# Autodesk Inventor assembly: 23-004
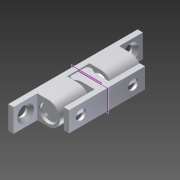
[picture p0: Inventor's stored thumbnail of the model, 180x180]
Saved by Autodesk Inventor 2013 SP1 (Build 170176100, 176)
## iProperties
Created: 2011-01-07
Part Number: 23-004
Document SubType Name: Assembly
Designer: dc85560
Stock Number: 23-004
Mass: 2.95223 g
Surface Area: 29.5918 cm^2
Volume: 2.95223 cm^3
Density: 1 g/cm^3
Translation Standard: STEP AP214IS
File Name: 0930462.STEP
Preprocessor: SolidWorks 2010
Postprocessor: Build: 320, Release: 2008 SP2 - Date: Mon 11/26/2007
Sent Units: MILLIMETERS
Uncertainty: 1e-05
Author: dc85560
## Documents named in this file (4)
- C:\Program Files\Autodesk\PSD 3.0\PSD 3 Library Update\IPS Part Files\05-Handles_Hinges\17-Catches\23-004.iam
- C:\Program Files\Autodesk\PSD 3.0\PSD 3 Library Update\IPS Part Files\05-Handles_Hinges\17-Catches\23-004Z1.ipt
- C:\Program Files\Autodesk\PSD 3.0\PSD 3 Library Update\IPS Part Files\05-Handles_Hinges\17-Catches\23-004Z3.ipt
- C:\Program Files\Autodesk\PSD 3.0\PSD 3 Library Update\IPS Part Files\05-Handles_Hinges\17-Catches\23-004Z2.ipt
## Components (4 placed, 3 different names)
1. 23-004Z1:1 — Flush:1, Tangent:1, Tangent:2, Flush:2
2. 23-004Z3:1 — Flush:1, Mate:1, Mate:2, Flush:2
3. 23-004Z2:1 — Mate:2, Tangent:1
4. 23-004Z2:2 — Mate:1, Tangent:2
## Relationships (6: Flush 2, Mate 2, Tangent 2)
- Flush:1 (0.6 mm): 23-004Z1:1 ↔ 23-004Z3:1
- Mate:1: 23-004Z3:1 ↔ 23-004Z2:2
- Mate:2: 23-004Z3:1 ↔ 23-004Z2:1
- Tangent:1: 23-004Z1:1 ↔ 23-004Z2:1
- Tangent:2: 23-004Z1:1 ↔ 23-004Z2:2
- Flush:2: 23-004Z1:1 ↔ 23-004Z3:1
